# Autodesk Inventor assembly: flute
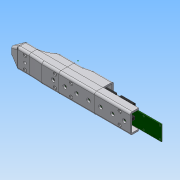
[picture p0: Inventor's stored thumbnail of the model, 180x180]
Saved by Autodesk Inventor 2015 (Build 190159000, 159)
## iProperties
Created: 2015-08-12
Part Number: flute
Document SubType Name: Assembly
Designer: Gregwar
Author: Gregwar
## Documents named in this file (9)
- C:\Users\Gregwar\Desktop\eFlute\3d\flute.iam
- C:\Users\Gregwar\Desktop\eFlute\3d\electronics.ipt
- C:\Users\Gregwar\Desktop\eFlute\3d\mouth.ipt
- C:\Users\Gregwar\Desktop\eFlute\3d\part1_top.ipt
- C:\Users\Gregwar\Desktop\eFlute\3d\part1_bottom.ipt
- C:\Users\Gregwar\Desktop\eFlute\3d\entretoise_12.ipt
- C:\Users\Gregwar\Desktop\eFlute\3d\part2_top.ipt
- C:\Users\Gregwar\Desktop\eFlute\3d\part2_bottom.ipt
- C:\Users\Gregwar\Desktop\eFlute\3d\part3_top.ipt
## Components (10 placed, 8 different names)
1. electronics:1 — Placage:1, Placage:2, Placage:3, Placage:5, Placage:7, Placage:9, Placage:10, Placage:11, Placage:12, Placage:15, Placage:17, Placage:24, Placage:25, Placage:29
2. mouth:1 — Placage:1, Placage:2, Placage:3, Placage:4, Placage:6
3. part1_top:1 — Placage:4, Placage:5, Placage:8, Placage:14
4. part1_bottom:1 — Placage:6, Placage:7, Placage:8, Placage:13, Placage:16
5. entretoise_12:1 — Placage:10, Placage:12
6. entretoise_12:2 — Placage:9, Placage:11, Placage:13
7. part2_top:1 — Placage:14, Placage:15, Placage:23, Placage:28
8. part2_bottom:1 — Placage:16, Placage:17, Placage:23, Placage:26, Placage:27
9. entretoise_12:3 — Placage:24, Placage:25, Placage:26, Placage:27
10. part3_top:1 — Placage:28, Placage:29
## Relationships (24: Mate 24)
- Placage:1 [Mate]: electronics:1 ↔ mouth:1
- Placage:2 [Mate]: electronics:1 ↔ mouth:1
- Placage:3 [Mate]: electronics:1 ↔ mouth:1
- Placage:4 [Mate]: mouth:1 ↔ part1_top:1
- Placage:5 [Mate]: electronics:1 ↔ part1_top:1
- Placage:6 [Mate]: mouth:1 ↔ part1_bottom:1
- Placage:7 [Mate]: electronics:1 ↔ part1_bottom:1
- Placage:8 [Mate]: part1_top:1 ↔ part1_bottom:1
- Placage:9 [Mate]: electronics:1 ↔ entretoise_12:2
- Placage:10 [Mate]: electronics:1 ↔ entretoise_12:1
- Placage:11 [Mate]: electronics:1 ↔ entretoise_12:2
- Placage:12 [Mate]: electronics:1 ↔ entretoise_12:1
- Placage:13 [Mate]: part1_bottom:1 ↔ entretoise_12:2
- Placage:14 [Mate]: part1_top:1 ↔ part2_top:1
- Placage:15 [Mate]: electronics:1 ↔ part2_top:1
- Placage:16 [Mate]: part1_bottom:1 ↔ part2_bottom:1
- Placage:17 [Mate]: electronics:1 ↔ part2_bottom:1
- Placage:23 [Mate]: part2_top:1 ↔ part2_bottom:1
- Placage:24 [Mate]: electronics:1 ↔ entretoise_12:3
- Placage:25 [Mate]: electronics:1 ↔ entretoise_12:3
- Placage:26 [Mate]: part2_bottom:1 ↔ entretoise_12:3
- Placage:27 [Mate]: part2_bottom:1 ↔ entretoise_12:3
- Placage:28 [Mate]: part2_top:1 ↔ part3_top:1
- Placage:29 [Mate]: electronics:1 ↔ part3_top:1
